# Autodesk Inventor assembly: Track Idler Assembly
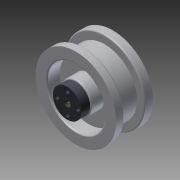
[picture p0: Inventor's stored thumbnail of the model, 180x180]
Saved by Autodesk Inventor 2015 (Build 190159000, 159)
## iProperties
Created: 2015-09-26
Part Number: Track Idler Assembly
Document SubType Name: Assembly
Designer: Jing-Chen
Author: Jing-Chen
## Documents named in this file (3)
- C:\Users\Jing-Chen\Desktop\Bionic Hybrids 2016\Bionic-Hybrids\CAD\Drivetrain\Sub-Assemblies\Track Idler Assembly.iam
- C:\Users\Jing-Chen\Desktop\Bionic Hybrids 2016\Bionic-Hybrids\Stock\Track Idler - 73646.ipt
- C:\Users\Jing-Chen\Desktop\Bionic Hybrids 2016\Bionic-Hybrids\Stock\Shaft Collar-Setscrew, Axle, Mountable - 739172.iam
## Components (2 placed, 2 different names)
1. Track Idler - 73646:1 — Mate:1, Mate:2, Mate:3
2. Shaft Collar-Setscrew, Axle, Mountable - 739172:1 [sub-assembly] — Mate:1, Mate:2, Mate:3
## Relationships (3: Mate 3)
- Mate:1: Track Idler - 73646:1 ↔ Shaft Collar-Setscrew, Axle, Mountable - 739172:1
- Mate:2: Track Idler - 73646:1 ↔ Shaft Collar-Setscrew, Axle, Mountable - 739172:1
- Mate:3: Track Idler - 73646:1 ↔ Shaft Collar-Setscrew, Axle, Mountable - 739172:1
